# Autodesk Inventor assembly: LiDAR
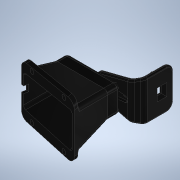
[picture p0: Inventor's stored thumbnail of the model, 180x180]
Saved by Autodesk Inventor 2020 (Build 240168000, 168)
## iProperties
Created: 2022-06-22
Part Number: LiDAR
Document SubType Name: Assembly
Designer: JCarlos
Author: JCarlos
## Documents named in this file (3)
- C:\Users\candu\Google Drive\Doutorado_UTFPR\Projeto_1_SpotMicro\Projeto_3D\Robo_Montado_v3\LiDAR.iam
- C:\Users\candu\Google Drive\Doutorado_UTFPR\Projeto_1_SpotMicro\Projeto_3D\Robo_Montado_v3\Base_Lidarv2.ipt
- C:\Users\candu\Google Drive\Doutorado_UTFPR\Projeto_1_SpotMicro\Projeto_3D\Robo_Montado_v3\Suporte_Laserv2.ipt
## Components (2 placed, 2 different names)
1. Base_Lidarv2:1 — Coincidência:1, Coincidência:2, Ângulo:1
2. Suporte_Laserv2:1 — Coincidência:1, Coincidência:2, Ângulo:1
## Relationships (3: Mate 2, Angle 1)
- Coincidência:1 [Mate]: Base_Lidarv2:1 ↔ Suporte_Laserv2:1
- Coincidência:2 [Mate] (1 mm): Base_Lidarv2:1 ↔ Suporte_Laserv2:1
- Ângulo:1 [Angle] (90 deg): Base_Lidarv2:1 ↔ Suporte_Laserv2:1
